# Autodesk Inventor assembly: Base
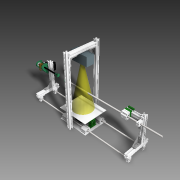
[picture p0: Inventor's stored thumbnail of the model, 180x180]
Saved by Autodesk Inventor 2015 (Build 190159000, 159)
## iProperties
Created: 2015-02-24
Part Number: Base
Document SubType Name: Assembly
Designer: Andrew
Author: Andrew
## Documents named in this file (29)
- C:\Users\pltwe4\Documents\model\Base.iam
- C:\Users\pltwe4\Documents\model\Linear Bearing Platform Small.ipt
- C:\Users\pltwe4\Documents\model\Base Plate.ipt
- C:\Users\pltwe4\Documents\model\NEMA 17 Stepper.ipt
- C:\Users\pltwe4\Documents\model\GT2 Pulley.ipt
- C:\Users\pltwe4\Documents\model\Stepper Motor Mount.ipt
- C:\Users\pltwe4\Documents\model\MainRod.ipt
- C:\Users\pltwe4\Documents\model\Linear Rail Shaft Guide.ipt
- C:\Users\pltwe4\Documents\model\Belt Tensioner Assy.iam
- C:\Users\pltwe4\Documents\model\Spur Gear.ipt
- C:\Users\pltwe4\Documents\model\Worm Gear.ipt
- C:\Users\pltwe4\Documents\model\20x20 Slotted Extrusion Arm.ipt
- C:\Users\pltwe4\Documents\model\20x20 Slotted Extrusion Tower.ipt
- C:\Users\pltwe4\Documents\model\Corner Brace.ipt
- C:\Users\pltwe4\Documents\model\Worm Gear Box.ipt
- C:\Users\pltwe4\Documents\model\Bearing.ipt
- C:\Users\pltwe4\Documents\model\20x20 Slotted Extrusion Stationary Arm.ipt
- C:\Users\pltwe4\Documents\model\Clamp Rod.ipt
- C:\Users\pltwe4\Documents\model\Rotational Rod.ipt
- C:\Users\pltwe4\Documents\model\20x20 Slotted Extrusion Base.ipt
- C:\Users\pltwe4\Documents\model\20x20 Slotted Extrusion Source Bracket.ipt
- C:\Users\pltwe4\Documents\model\Exposure.ipt
- C:\Users\pltwe4\Documents\model\Cover.ipt
- C:\Users\pltwe4\Documents\model\Tensioning Bracket.ipt
- C:\Users\pltwe4\Documents\model\Linear Bearing Platform Adapter Back.ipt
- C:\Users\pltwe4\Documents\model\Linear Bearing Platform Adapter.ipt
- C:\Users\pltwe4\Documents\model\X-Ray Tube Assy.ipt.iam
- C:\Users\pltwe4\Documents\model\Hand.ipt
- X-Ray Tube Assy.ipt
## Components (52 placed, 27 different names)
1. Linear Bearing Platform Small:1 — Flush:5, Mate:7, Flush:9, Flush:11, Flush:12
2. Linear Bearing Platform Small:2 — Flush:4, Flush:5, Flush:6, Mate:6, Angle:2, Flush:8, Flush:10
3. Linear Bearing Platform Small:3 — Flush:4, Mate:8, Flush:8
4. Linear Bearing Platform Small:4 — Flush:6, Mate:1, Mate:9, Angle:3, Flush:9, Flush:13
5. Base Plate:1 — Flush:1, Flush:2, Flush:3, Mate:1, Mate:5, Angle:2, Angle:3, Flush:10, Flush:11, Flush:12, Flush:13, Angle:4, Flush:26, Flush:27, Mate:24, Flush:30, Mate:104, Mate:105, Flush:40, Flush:42, Mate:123, Flush:43, Mate:127
6. NEMA 17 Stepper:1 — Mate:4, Flush:7, Angle:1, Mate:14, Mate:15
7. GT2 Pulley:1 — Mate:4, Flush:7, Mate:22, Mate:112
8. Stepper Motor Mount:1 — Angle:1, Mate:5, Angle:4, Mate:14, Mate:15, Flush:30
9. MainRod:1 — Mate:6, Mate:7, Mate:10, Flush:16, Mate:12, Flush:24
10. MainRod:2 — Mate:8, Mate:9, Mate:11, Flush:16, Mate:13, Flush:23
11. Linear Rail Shaft Guide:1 — Mate:10, Flush:14, Flush:15, Flush:24
12. Linear Rail Shaft Guide:2 — Mate:11, Flush:14, Flush:15, Flush:31, Mate:47, Mate:48
13. Linear Rail Shaft Guide:3 — Mate:12
14. Linear Rail Shaft Guide:4 — Mate:13, Flush:23, Flush:32, Mate:49, Mate:50
15. Belt Tensioner Assy:1 [sub-assembly] — Flush:25, Mate:23, Symmetry:1, Mate:124, Mate:126
16. Belt Tensioner Assy:2 [sub-assembly] — Flush:25, Symmetry:1, Mate:125, Mate:129
17. Base Plate:2 — Flush:26, Flush:27, Mate:24
18. Spur Gear:1 — Tangent:1, Mate:44, Mate:46, Angle:5, Mate:87, Mate:99
19. Stepper Motor Mount:2 — Mate:40, Mate:41, Mate:42, Angle:5, Mate:53, Mate:54, Mate:55, Mate:79
20. Worm Gear:1 — Mate:27, Mate:28, Tangent:1, Mate:44, Mate:46, Mate:80
21. NEMA 17 Stepper:2 — Mate:27, Mate:28, Mate:40, Mate:41, Mate:42, Mate:81
22. 20x20 Slotted Extrusion Arm:1 — Flush:31, Mate:47, Mate:48, Mate:52, Flush:34, Mate:66, Mate:68, Mate:70, Mate:72, Mate:100
23. 20x20 Slotted Extrusion Tower:1 — Mate:52, Flush:34, Mate:53, Mate:54, Mate:55, Mate:65, Mate:67, Mate:69, Mate:71
24. 20x20 Slotted Extrusion Arm:2 — Flush:32, Mate:49, Mate:50, Mate:51, Flush:33, Mate:57, Mate:58, Mate:63, Mate:64
25. 20x20 Slotted Extrusion Tower:2 — Mate:51, Flush:33, Mate:59, Mate:60, Mate:61, Mate:62, Angle:7, Mate:88, Mate:89, Mate:90, Flush:35, Flush:36, Mate:92, Mate:95
26. Corner Brace:1 — Mate:69, Mate:70, Mate:71, Mate:72
27. Corner Brace:2 — Mate:65, Mate:66, Mate:67, Mate:68
28. Corner Brace:3 — Mate:57, Mate:58, Mate:59, Mate:60
29. Corner Brace:4 — Mate:61, Mate:62, Mate:63, Mate:64
30. Linear Bearing Platform Small:5 — Mate:86, Angle:6, Mate:87, Mate:91, Mate:93, Mate:130, Mate:131, Mate:132
31. Linear Rail Shaft Guide:5 — Mate:86, Angle:6, Angle:7, Mate:88, Mate:89, Mate:90, Flush:35, Mate:91, Flush:50
32. Worm Gear Box:1 — Mate:79, Mate:80, Mate:81, Mate:82, Mate:84, Flush:37
33. Bearing:1 — Mate:82
34. Bearing:2 — Mate:84
35. 20x20 Slotted Extrusion Stationary Arm:1 — Flush:36, Mate:92, Mate:93, Mate:94, Mate:96, Mate:97, Mate:133
36. Corner Brace:5 — Mate:94, Mate:95, Mate:96, Mate:97
37. Clamp Rod:1 — Mate:98, Flush:50, Mate:147
38. Rotational Rod:1 — Mate:98, Mate:99, Flush:37, Mate:100, Mate:112, Mate:146, Mate:148
39. 20x20 Slotted Extrusion Base:1 — Mate:104, Symmetry:2, Flush:39, Mate:106, Flush:40, Mate:135, Mate:137
40. 20x20 Slotted Extrusion Base:2 — Mate:105, Symmetry:2, Flush:39, Mate:106, Mate:107, Flush:41, Mate:134
41. 20x20 Slotted Extrusion Source Bracket:1 — Mate:107, Flush:41, Mate:140, Mate:141, Mate:142, Mate:143, Mate:144
42. Exposure:1 — Mate:138, Mate:139
43. Cover:1 — Flush:42, Mate:123, Flush:43
44. Tensioning Bracket:1 — Flush:44, Flush:45, Mate:125, Mate:126, Mate:128, Mate:129
45. Tensioning Bracket:2 — Flush:44, Flush:45, Mate:124, Mate:127, Mate:128
46. Linear Bearing Platform Adapter Back:1 — Flush:46, Flush:47, Mate:133
47. Linear Bearing Platform Adapter:1 — Flush:46, Flush:47, Mate:130, Mate:131, Mate:132
48. Corner Brace:6 — Mate:135, Flush:48, Flush:49, Mate:137
49. Corner Brace:7 — Mate:134, Flush:48, Flush:49, Mate:144
50. X-Ray Tube Assy.ipt:1 [sub-assembly] — Mate:138, Mate:139, Mate:140, Mate:141, Mate:142, Mate:143
51. Hand:1 — Mate:145, Mate:146, Mate:148
52. Hand:2 — Mate:145, Mate:147
## Relationships (151: Mate 98, Flush 43, Angle 7, Symmetry 2, Tangent 1)
- Flush:1: Base Plate:1
- Flush:2: Base Plate:1
- Flush:3: Base Plate:1
- Flush:4: Linear Bearing Platform Small:2 ↔ Linear Bearing Platform Small:3
- Flush:5: Linear Bearing Platform Small:1 ↔ Linear Bearing Platform Small:2
- Flush:6: Linear Bearing Platform Small:2 ↔ Linear Bearing Platform Small:4
- Mate:1: Linear Bearing Platform Small:4 ↔ Base Plate:1
- Mate:4: NEMA 17 Stepper:1 ↔ GT2 Pulley:1
- Flush:7: NEMA 17 Stepper:1 ↔ GT2 Pulley:1
- Angle:1 (0 deg): NEMA 17 Stepper:1 ↔ Stepper Motor Mount:1
- Mate:5 (10 mm): Base Plate:1 ↔ Stepper Motor Mount:1
- Mate:6: Linear Bearing Platform Small:2 ↔ MainRod:1
- Mate:7: Linear Bearing Platform Small:1 ↔ MainRod:1
- Mate:8: Linear Bearing Platform Small:3 ↔ MainRod:2
- Mate:9: Linear Bearing Platform Small:4 ↔ MainRod:2
- Mate:10: MainRod:1 ↔ Linear Rail Shaft Guide:1
- Mate:11: MainRod:2 ↔ Linear Rail Shaft Guide:2
- Angle:2 (0 deg): Linear Bearing Platform Small:2 ↔ Base Plate:1
- Angle:3 (0 deg): Linear Bearing Platform Small:4 ↔ Base Plate:1
- Flush:8: Linear Bearing Platform Small:2 ↔ Linear Bearing Platform Small:3
- Flush:9: Linear Bearing Platform Small:1 ↔ Linear Bearing Platform Small:4
- Flush:10 (5 mm): Linear Bearing Platform Small:2 ↔ Base Plate:1
- Flush:11 (5 mm): Linear Bearing Platform Small:1 ↔ Base Plate:1
- Flush:12 (5 mm): Linear Bearing Platform Small:1 ↔ Base Plate:1
- Flush:13 (5 mm): Linear Bearing Platform Small:4 ↔ Base Plate:1
- Flush:14: Linear Rail Shaft Guide:1 ↔ Linear Rail Shaft Guide:2
- Flush:15: Linear Rail Shaft Guide:1 ↔ Linear Rail Shaft Guide:2
- Flush:16: MainRod:1 ↔ MainRod:2
- Angle:4 (180 deg): Base Plate:1 ↔ Stepper Motor Mount:1
- [Flush]: Linear Rail Shaft Guide:3 ↔ Linear Rail Shaft Guide:4
- [Flush]: Linear Rail Shaft Guide:3 ↔ Linear Rail Shaft Guide:4
- Mate:12: MainRod:1 ↔ Linear Rail Shaft Guide:3
- Mate:13: MainRod:2 ↔ Linear Rail Shaft Guide:4
- Mate:14: NEMA 17 Stepper:1 ↔ Stepper Motor Mount:1
- Mate:15: NEMA 17 Stepper:1 ↔ Stepper Motor Mount:1
- Flush:23 (5 mm): MainRod:2 ↔ Linear Rail Shaft Guide:4
- Flush:24 (5 mm): MainRod:1 ↔ Linear Rail Shaft Guide:1
- Mate:22: GT2 Pulley:1
- Flush:25: Belt Tensioner Assy:1 ↔ Belt Tensioner Assy:2
- Mate:23: Belt Tensioner Assy:1
- Flush:26: Base Plate:1 ↔ Base Plate:2
- Flush:27: Base Plate:1 ↔ Base Plate:2
- Mate:24 (65 mm): Base Plate:1 ↔ Base Plate:2
- Mate:27: Worm Gear:1 ↔ NEMA 17 Stepper:2
- Mate:28 (3 mm): Worm Gear:1 ↔ NEMA 17 Stepper:2
- Flush:30: Base Plate:1 ↔ Stepper Motor Mount:1
- Mate:40: Stepper Motor Mount:2 ↔ NEMA 17 Stepper:2
- Mate:41: Stepper Motor Mount:2 ↔ NEMA 17 Stepper:2
- Mate:42: Stepper Motor Mount:2 ↔ NEMA 17 Stepper:2
- Tangent:1: Spur Gear:1 ↔ Worm Gear:1
- Mate:44: Spur Gear:1 ↔ Worm Gear:1
- Mate:46: Spur Gear:1 ↔ Worm Gear:1
- Angle:5 (0 deg): Spur Gear:1 ↔ Stepper Motor Mount:2
- Flush:31: Linear Rail Shaft Guide:2 ↔ 20x20 Slotted Extrusion Arm:1
- Mate:47: Linear Rail Shaft Guide:2 ↔ 20x20 Slotted Extrusion Arm:1
- Mate:48: Linear Rail Shaft Guide:2 ↔ 20x20 Slotted Extrusion Arm:1
- Flush:32: Linear Rail Shaft Guide:4 ↔ 20x20 Slotted Extrusion Arm:2
- Mate:49: Linear Rail Shaft Guide:4 ↔ 20x20 Slotted Extrusion Arm:2
- Mate:50: Linear Rail Shaft Guide:4 ↔ 20x20 Slotted Extrusion Arm:2
- Mate:51: 20x20 Slotted Extrusion Arm:2 ↔ 20x20 Slotted Extrusion Tower:2
- Flush:33: 20x20 Slotted Extrusion Arm:2 ↔ 20x20 Slotted Extrusion Tower:2
- Mate:52: 20x20 Slotted Extrusion Arm:1 ↔ 20x20 Slotted Extrusion Tower:1
- Flush:34: 20x20 Slotted Extrusion Arm:1 ↔ 20x20 Slotted Extrusion Tower:1
- Mate:53: Stepper Motor Mount:2 ↔ 20x20 Slotted Extrusion Tower:1
- Mate:54: Stepper Motor Mount:2 ↔ 20x20 Slotted Extrusion Tower:1
- Mate:55: Stepper Motor Mount:2 ↔ 20x20 Slotted Extrusion Tower:1
- Mate:57: 20x20 Slotted Extrusion Arm:2 ↔ Corner Brace:3
- Mate:58: 20x20 Slotted Extrusion Arm:2 ↔ Corner Brace:3
- Mate:59: 20x20 Slotted Extrusion Tower:2 ↔ Corner Brace:3
- Mate:60: 20x20 Slotted Extrusion Tower:2 ↔ Corner Brace:3
- Mate:61: 20x20 Slotted Extrusion Tower:2 ↔ Corner Brace:4
- Mate:62: 20x20 Slotted Extrusion Tower:2 ↔ Corner Brace:4
- Mate:63: 20x20 Slotted Extrusion Arm:2 ↔ Corner Brace:4
- Mate:64: 20x20 Slotted Extrusion Arm:2 ↔ Corner Brace:4
- Mate:65: 20x20 Slotted Extrusion Tower:1 ↔ Corner Brace:2
- Mate:66: 20x20 Slotted Extrusion Arm:1 ↔ Corner Brace:2
- Mate:67: 20x20 Slotted Extrusion Tower:1 ↔ Corner Brace:2
- Mate:68: 20x20 Slotted Extrusion Arm:1 ↔ Corner Brace:2
- Mate:69: 20x20 Slotted Extrusion Tower:1 ↔ Corner Brace:1
- Mate:70: 20x20 Slotted Extrusion Arm:1 ↔ Corner Brace:1
- Mate:71: 20x20 Slotted Extrusion Tower:1 ↔ Corner Brace:1
- Mate:72: 20x20 Slotted Extrusion Arm:1 ↔ Corner Brace:1
- Mate:79: Stepper Motor Mount:2 ↔ Worm Gear Box:1
- Mate:80: Worm Gear:1 ↔ Worm Gear Box:1
- Mate:81: NEMA 17 Stepper:2 ↔ Worm Gear Box:1
- Mate:82: Worm Gear Box:1 ↔ Bearing:1
- Mate:84: Worm Gear Box:1 ↔ Bearing:2
- Mate:86: Linear Bearing Platform Small:5 ↔ Linear Rail Shaft Guide:5
- Angle:6 (0 deg): Linear Bearing Platform Small:5 ↔ Linear Rail Shaft Guide:5
- Angle:7 (0 deg): 20x20 Slotted Extrusion Tower:2 ↔ Linear Rail Shaft Guide:5
- Mate:87: Spur Gear:1 ↔ Linear Bearing Platform Small:5
- Mate:88: 20x20 Slotted Extrusion Tower:2 ↔ Linear Rail Shaft Guide:5
- Mate:89: 20x20 Slotted Extrusion Tower:2 ↔ Linear Rail Shaft Guide:5
- Mate:90: 20x20 Slotted Extrusion Tower:2 ↔ Linear Rail Shaft Guide:5
- Flush:35 (-5 mm): 20x20 Slotted Extrusion Tower:2 ↔ Linear Rail Shaft Guide:5
- Mate:91 (50 mm): Linear Bearing Platform Small:5 ↔ Linear Rail Shaft Guide:5
- Flush:36: 20x20 Slotted Extrusion Tower:2 ↔ 20x20 Slotted Extrusion Stationary Arm:1
- Mate:92: 20x20 Slotted Extrusion Tower:2 ↔ 20x20 Slotted Extrusion Stationary Arm:1
- Mate:93: Linear Bearing Platform Small:5 ↔ 20x20 Slotted Extrusion Stationary Arm:1
- Mate:94: 20x20 Slotted Extrusion Stationary Arm:1 ↔ Corner Brace:5
- Mate:95: 20x20 Slotted Extrusion Tower:2 ↔ Corner Brace:5
- Mate:96: 20x20 Slotted Extrusion Stationary Arm:1 ↔ Corner Brace:5
- Mate:97: 20x20 Slotted Extrusion Stationary Arm:1 ↔ Corner Brace:5
- Mate:98: Clamp Rod:1 ↔ Rotational Rod:1
- Mate:99: Spur Gear:1 ↔ Rotational Rod:1
- Flush:37 (-5 mm): Worm Gear Box:1 ↔ Rotational Rod:1
- Mate:100: 20x20 Slotted Extrusion Arm:1 ↔ Rotational Rod:1
- Symmetry:1: Belt Tensioner Assy:1 ↔ Belt Tensioner Assy:2
- Mate:104: Base Plate:1 ↔ 20x20 Slotted Extrusion Base:1
- Mate:105: Base Plate:1 ↔ 20x20 Slotted Extrusion Base:2
- Symmetry:2: 20x20 Slotted Extrusion Base:1 ↔ 20x20 Slotted Extrusion Base:2
- Flush:39: 20x20 Slotted Extrusion Base:1 ↔ 20x20 Slotted Extrusion Base:2
- Mate:106 (150 mm): 20x20 Slotted Extrusion Base:1 ↔ 20x20 Slotted Extrusion Base:2
- Flush:40: Base Plate:1 ↔ 20x20 Slotted Extrusion Base:1
- Mate:107: 20x20 Slotted Extrusion Base:2 ↔ 20x20 Slotted Extrusion Source Bracket:1
- Flush:41: 20x20 Slotted Extrusion Base:2 ↔ 20x20 Slotted Extrusion Source Bracket:1
- Mate:112: GT2 Pulley:1 ↔ Rotational Rod:1
- Flush:42: Base Plate:1 ↔ Cover:1
- Mate:123: Base Plate:1 ↔ Cover:1
- Flush:43: Base Plate:1 ↔ Cover:1
- Flush:44: Tensioning Bracket:1 ↔ Tensioning Bracket:2
- Flush:45: Tensioning Bracket:1 ↔ Tensioning Bracket:2
- Mate:124: Belt Tensioner Assy:1 ↔ Tensioning Bracket:2
- Mate:125: Belt Tensioner Assy:2 ↔ Tensioning Bracket:1
- Mate:126: Belt Tensioner Assy:1 ↔ Tensioning Bracket:1
- Mate:127: Base Plate:1 ↔ Tensioning Bracket:2
- Mate:128 (100 mm): Tensioning Bracket:1 ↔ Tensioning Bracket:2
- Mate:129 (25 mm): Belt Tensioner Assy:2 ↔ Tensioning Bracket:1
- Flush:46: Linear Bearing Platform Adapter Back:1 ↔ Linear Bearing Platform Adapter:1
- Flush:47: Linear Bearing Platform Adapter Back:1 ↔ Linear Bearing Platform Adapter:1
- Mate:130: Linear Bearing Platform Small:5 ↔ Linear Bearing Platform Adapter:1
- Mate:131: Linear Bearing Platform Small:5 ↔ Linear Bearing Platform Adapter:1
- Mate:132: Linear Bearing Platform Small:5 ↔ Linear Bearing Platform Adapter:1
- Mate:133: 20x20 Slotted Extrusion Stationary Arm:1 ↔ Linear Bearing Platform Adapter Back:1
- Mate:134: 20x20 Slotted Extrusion Base:2 ↔ Corner Brace:7
- Mate:135: 20x20 Slotted Extrusion Base:1 ↔ Corner Brace:6
- Flush:48: Corner Brace:6 ↔ Corner Brace:7
- Flush:49: Corner Brace:6 ↔ Corner Brace:7
- Mate:137: 20x20 Slotted Extrusion Base:1 ↔ Corner Brace:6
- Mate:138: Exposure:1 ↔ X-Ray Tube Assy.ipt:1
- Mate:139: Exposure:1 ↔ X-Ray Tube Assy.ipt:1
- Mate:140: 20x20 Slotted Extrusion Source Bracket:1 ↔ X-Ray Tube Assy.ipt:1
- Mate:141: 20x20 Slotted Extrusion Source Bracket:1 ↔ X-Ray Tube Assy.ipt:1
- Mate:142: 20x20 Slotted Extrusion Source Bracket:1 ↔ X-Ray Tube Assy.ipt:1
- Mate:143: 20x20 Slotted Extrusion Source Bracket:1 ↔ X-Ray Tube Assy.ipt:1
- Mate:144: 20x20 Slotted Extrusion Source Bracket:1 ↔ Corner Brace:7
- Flush:50 (100 mm): Linear Rail Shaft Guide:5 ↔ Clamp Rod:1
- Mate:145: Hand:1 ↔ Hand:2
- Mate:146: Rotational Rod:1 ↔ Hand:1
- Mate:147: Clamp Rod:1 ↔ Hand:2
- Mate:148: Rotational Rod:1 ↔ Hand:1
## Named parameters: d31_d27 = 0 mm, d32_d28 = 0 mm
